# Autodesk Inventor assembly: YCart
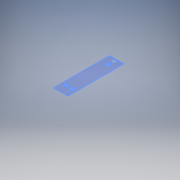
[picture p0: Inventor's stored thumbnail of the model, 180x180]
Saved by Autodesk Inventor 2019 (Build 230136000, 136)
## iProperties
Created: 2019-08-21
Part Number: YCart
Document SubType Name: Assembly
Designer: Bruno
Author: Bruno
## Documents named in this file (3)
- C:\Users\Bruno\Stuff\TPINFO\tp-info\YCart.iam
- C:\Users\Bruno\Stuff\TPINFO\tp-info\YCartFloor.ipt
- C:\Users\Bruno\Stuff\TPINFO\tp-info\Lm8uu.ipt
## Components (3 placed, 2 different names)
1. YCartFloor:1 — Rigid:1, Rigid:2
2. Lm8uu:1 — Rigid:1
3. Lm8uu:2 — Rigid:2
## Relationships (2: WeldJoint 2)
- Rigid:1 [WeldJoint]: YCartFloor:1 ↔ Lm8uu:1
- Rigid:2 [WeldJoint]: YCartFloor:1 ↔ Lm8uu:2
